# Autodesk Inventor assembly: Wrist
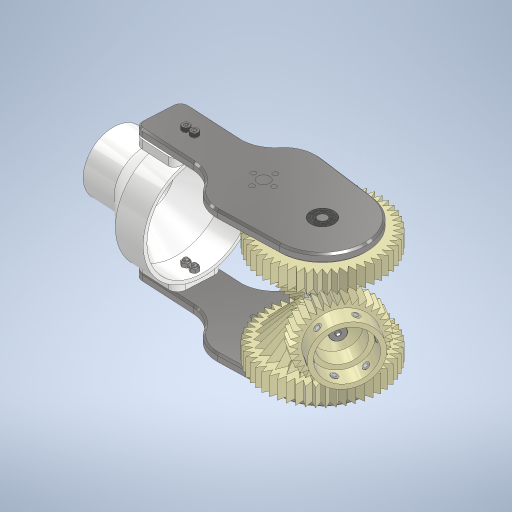
[picture p0: Inventor's stored thumbnail of the model, 512x512]
Saved by Autodesk Inventor 2023 (Build 270158030, 158C)
## iProperties
Created: 2022-09-21
Part Number: Wrist
Document SubType Name: Assembly
Designer: caden
Author: caden
## Documents named in this file (16)
- V:\Robtotics\Wrist\Wrist.iam
- V:\Robtotics\Wrist\Wrist Side Brase.ipt
- V:\Robtotics\2in to 4in Reducer.ipt
- V:\Robtotics\Wrist\Pipe Holder.ipt
- V:\Robtotics\Hardware\1265K77_Rotary Shaft.ipt
- V:\Robtotics\Hardware\2349K412_Permanently Lubricated Ball Bearing.ipt
- V:\Robtotics\Wrist\Bevel Gear.ipt
- V:\Robtotics\Wrist\Shim.ipt
- V:\Robtotics\Wrist\Space.ipt
- V:\Robtotics\Wrist\Bevel Middle.ipt
- V:\Robtotics\Hardware\92981A305_Alloy Steel Shoulder Screws.ipt
- V:\Robtotics\Wrist\Bevel Gear Opposite.ipt
- V:\Robtotics\Hardware\91290A252_NO THREADS_Alloy Steel Socket Head Screw.ipt
- V:\Robtotics\Hardware\94645A102_NO THREADS_High-Strength Steel Nylon-Insert Locknut.ipt
- V:\Robtotics\Hardware\91290A047_NO THREADS_Black-Oxide Alloy Steel Socket Head Screw.ipt
- V:\Robtotics\Hardware\94180A361_NO THREADS_Tapered Heat-Set Inserts for Plastic.ipt
## Components (39 placed, 15 different names)
1. Wrist Side Brase:1 — Mate:1, Mate:3, Mate:15, Rotational:2, Rotational:3, Rotational:10, Mate:33, Mate:34, Mate:35
2. Wrist Side Brase:2 — Mate:1, Mate:3, Mate:15, Rotational:1, Rotational:4, Mate:21, Rotational:9, Mate:36, Mate:37
3. 2in to 4in Reducer:1 — Flush:3, Mate:21
4. Pipe Holder:1 — Mate:33, Mate:34, Mate:35
5. Pipe Holder:2 — Flush:3, Mate:36, Mate:37
6. 1265K77_Rotary Shaft:1 — Rotational:1, Rotational:2, Mate:24, Rotational:11
7. 2349K412_Permanently Lubricated Ball Bearing:1 — Rotational:3
8. 2349K412_Permanently Lubricated Ball Bearing:2 — Rotational:4
9. Bevel Gear:1 — Rotational:5, Rotational:6, Rotation:2
10. Bevel Gear:2 — Rotational:7, Rotational:8, Rotation:1, Rotation:3
11. 2349K412_Permanently Lubricated Ball Bearing:3 — Rotational:6, Rotational:9
12. 2349K412_Permanently Lubricated Ball Bearing:4 — Rotational:5
13. 2349K412_Permanently Lubricated Ball Bearing:5 — Rotational:8, Rotational:10
14. 2349K412_Permanently Lubricated Ball Bearing:6 — Rotational:7
15. Shim:1 — Mate:23
16. Shim:2 — Mate:22
17. Space:1 — Mate:22, Mate:23, Mate:24, Rotational:11, Mate:50, Mate:51, Mate:52, Mate:53
18. 92981A305_Alloy Steel Shoulder Screws:1 — Rotational:13
19. 92981A305_Alloy Steel Shoulder Screws:2 — Rotational:12
20. Bevel Middle:1 — Mate:29, Mate:30, Rotational:12, Rotation:1, Rotation:2, Mate:54, Tangent:1
21. 2349K412_Permanently Lubricated Ball Bearing:7 — Mate:29, Mate:30
22. Bevel Gear Opposite:1 — Mate:31, Mate:32, Rotational:13, Rotation:3
23. 2349K412_Permanently Lubricated Ball Bearing:8 — Mate:31, Mate:32
24. 91290A252_NO THREADS_Alloy Steel Socket Head Screw:1 — Mate:49, Flush:7
25. 91290A252_NO THREADS_Alloy Steel Socket Head Screw:2 — Mate:46, Flush:4
26. 91290A252_NO THREADS_Alloy Steel Socket Head Screw:3 — Mate:48, Flush:6
27. 91290A252_NO THREADS_Alloy Steel Socket Head Screw:4 — Mate:47, Flush:5
28. 94645A102_NO THREADS_High-Strength Steel Nylon-Insert Locknut:1 — Mate:46, Flush:4
29. 94645A102_NO THREADS_High-Strength Steel Nylon-Insert Locknut:2 — Mate:49, Flush:7
30. 94645A102_NO THREADS_High-Strength Steel Nylon-Insert Locknut:3 — Mate:48, Flush:6
31. 94645A102_NO THREADS_High-Strength Steel Nylon-Insert Locknut:4 — Mate:47, Flush:5
32. 91290A047_NO THREADS_Black-Oxide Alloy Steel Socket Head Screw:1 — Mate:52, Mate:53
33. 91290A047_NO THREADS_Black-Oxide Alloy Steel Socket Head Screw:2 — Mate:50, Mate:51
34. 94180A361_NO THREADS_Tapered Heat-Set Inserts for Plastic:1 — Mate:54, Tangent:1
35. 94180A361_NO THREADS_Tapered Heat-Set Inserts for Plastic:2
36. 94180A361_NO THREADS_Tapered Heat-Set Inserts for Plastic:3
37. 94180A361_NO THREADS_Tapered Heat-Set Inserts for Plastic:4
38. 94180A361_NO THREADS_Tapered Heat-Set Inserts for Plastic:5
39. 94180A361_NO THREADS_Tapered Heat-Set Inserts for Plastic:6
## Component patterns: (6 elements, first: 94180A361_NO THREADS_Tapered Heat-Set Inserts for Plastic:1)
## Relationships (59: Mate 37, RevoluteJoint 13, Flush 5, RelateRotation 3, Tangent 1)
- Mate:1 (130 mm): Wrist Side Brase:1 ↔ Wrist Side Brase:2
- Mate:3: Wrist Side Brase:1 ↔ Wrist Side Brase:2
- Mate:15: Wrist Side Brase:1 ↔ Wrist Side Brase:2
- Flush:3: 2in to 4in Reducer:1 ↔ Pipe Holder:2
- Rotational:1 [RevoluteJoint]: Wrist Side Brase:2 ↔ 1265K77_Rotary Shaft:1
- Rotational:2 [RevoluteJoint]: Wrist Side Brase:1 ↔ 1265K77_Rotary Shaft:1
- Rotational:3 [RevoluteJoint]: Wrist Side Brase:1 ↔ 2349K412_Permanently Lubricated Ball Bearing:1
- Rotational:4 [RevoluteJoint]: Wrist Side Brase:2 ↔ 2349K412_Permanently Lubricated Ball Bearing:2
- Mate:21: Wrist Side Brase:2 ↔ 2in to 4in Reducer:1
- Rotational:5 [RevoluteJoint]: Bevel Gear:1 ↔ 2349K412_Permanently Lubricated Ball Bearing:4
- Rotational:6 [RevoluteJoint]: Bevel Gear:1 ↔ 2349K412_Permanently Lubricated Ball Bearing:3
- Rotational:7 [RevoluteJoint]: Bevel Gear:2 ↔ 2349K412_Permanently Lubricated Ball Bearing:6
- Rotational:8 [RevoluteJoint]: Bevel Gear:2 ↔ 2349K412_Permanently Lubricated Ball Bearing:5
- Rotational:9 [RevoluteJoint]: Wrist Side Brase:2 ↔ 2349K412_Permanently Lubricated Ball Bearing:3
- Rotational:10 [RevoluteJoint]: Wrist Side Brase:1 ↔ 2349K412_Permanently Lubricated Ball Bearing:5
- Mate:22: Shim:2 ↔ Space:1
- Mate:23: Shim:1 ↔ Space:1
- Mate:24: 1265K77_Rotary Shaft:1 ↔ Space:1
- Rotational:11 [RevoluteJoint]: 1265K77_Rotary Shaft:1 ↔ Space:1
- [Mate]: Space:1 ↔ 92981A305_Alloy Steel Shoulder Screws:1
- [Mate] (-13 mm): Space:1 ↔ 92981A305_Alloy Steel Shoulder Screws:1
- [Mate]: Space:1 ↔ 92981A305_Alloy Steel Shoulder Screws:2
- [Mate] (-13 mm): Space:1 ↔ 92981A305_Alloy Steel Shoulder Screws:2
- Mate:29: Bevel Middle:1 ↔ 2349K412_Permanently Lubricated Ball Bearing:7
- Mate:30: Bevel Middle:1 ↔ 2349K412_Permanently Lubricated Ball Bearing:7
- Rotational:12 [RevoluteJoint] (-3 mm): 92981A305_Alloy Steel Shoulder Screws:2 ↔ Bevel Middle:1
- Rotation:1 [RelateRotation] (1 ul): Bevel Gear:2 ↔ Bevel Middle:1
- Rotation:2 [RelateRotation] (1 ul): Bevel Gear:1 ↔ Bevel Middle:1
- Mate:31: Bevel Gear Opposite:1 ↔ 2349K412_Permanently Lubricated Ball Bearing:8
- Mate:32: Bevel Gear Opposite:1 ↔ 2349K412_Permanently Lubricated Ball Bearing:8
- Rotational:13 [RevoluteJoint] (-5 mm): 92981A305_Alloy Steel Shoulder Screws:1 ↔ Bevel Gear Opposite:1
- Rotation:3 [RelateRotation] (1 ul): Bevel Gear:2 ↔ Bevel Gear Opposite:1
- Mate:33: Wrist Side Brase:1 ↔ Pipe Holder:1
- Mate:34: Wrist Side Brase:1 ↔ Pipe Holder:1
- Mate:35: Wrist Side Brase:1 ↔ Pipe Holder:1
- Mate:36: Wrist Side Brase:2 ↔ Pipe Holder:2
- Mate:37: Wrist Side Brase:2 ↔ Pipe Holder:2
- [Mate]: Wrist Side Brase:2 ↔ 91290A252_NO THREADS_Alloy Steel Socket Head Screw:4
- [Mate]: Wrist Side Brase:2 ↔ 91290A252_NO THREADS_Alloy Steel Socket Head Screw:4
- [Mate]: Wrist Side Brase:2 ↔ 91290A252_NO THREADS_Alloy Steel Socket Head Screw:2
- [Mate]: Wrist Side Brase:2 ↔ 91290A252_NO THREADS_Alloy Steel Socket Head Screw:2
- [Mate]: Wrist Side Brase:1 ↔ 91290A252_NO THREADS_Alloy Steel Socket Head Screw:1
- [Mate]: Wrist Side Brase:1 ↔ 91290A252_NO THREADS_Alloy Steel Socket Head Screw:1
- [Mate]: Wrist Side Brase:1 ↔ 91290A252_NO THREADS_Alloy Steel Socket Head Screw:3
- [Mate]: Wrist Side Brase:1 ↔ 91290A252_NO THREADS_Alloy Steel Socket Head Screw:3
- Mate:46: 91290A252_NO THREADS_Alloy Steel Socket Head Screw:2 ↔ 94645A102_NO THREADS_High-Strength Steel Nylon-Insert Locknut:1
- Flush:4 (-2 mm): 91290A252_NO THREADS_Alloy Steel Socket Head Screw:2 ↔ 94645A102_NO THREADS_High-Strength Steel Nylon-Insert Locknut:1
- Mate:47: 91290A252_NO THREADS_Alloy Steel Socket Head Screw:4 ↔ 94645A102_NO THREADS_High-Strength Steel Nylon-Insert Locknut:4
- Flush:5 (-2 mm): 91290A252_NO THREADS_Alloy Steel Socket Head Screw:4 ↔ 94645A102_NO THREADS_High-Strength Steel Nylon-Insert Locknut:4
- Mate:48: 91290A252_NO THREADS_Alloy Steel Socket Head Screw:3 ↔ 94645A102_NO THREADS_High-Strength Steel Nylon-Insert Locknut:3
- Flush:6 (2 mm): 91290A252_NO THREADS_Alloy Steel Socket Head Screw:3 ↔ 94645A102_NO THREADS_High-Strength Steel Nylon-Insert Locknut:3
- Mate:49: 91290A252_NO THREADS_Alloy Steel Socket Head Screw:1 ↔ 94645A102_NO THREADS_High-Strength Steel Nylon-Insert Locknut:2
- Flush:7 (-2 mm): 91290A252_NO THREADS_Alloy Steel Socket Head Screw:1 ↔ 94645A102_NO THREADS_High-Strength Steel Nylon-Insert Locknut:2
- Mate:50: Space:1 ↔ 91290A047_NO THREADS_Black-Oxide Alloy Steel Socket Head Screw:2
- Mate:51: Space:1 ↔ 91290A047_NO THREADS_Black-Oxide Alloy Steel Socket Head Screw:2
- Mate:52: Space:1 ↔ 91290A047_NO THREADS_Black-Oxide Alloy Steel Socket Head Screw:1
- Mate:53: Space:1 ↔ 91290A047_NO THREADS_Black-Oxide Alloy Steel Socket Head Screw:1
- Mate:54: Bevel Middle:1 ↔ 94180A361_NO THREADS_Tapered Heat-Set Inserts for Plastic:1
- Tangent:1: Bevel Middle:1 ↔ 94180A361_NO THREADS_Tapered Heat-Set Inserts for Plastic:1
